# Autodesk Inventor assembly: złożenie ujoint
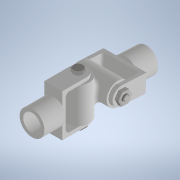
[picture p0: Inventor's stored thumbnail of the model, 180x180]
Saved by Autodesk Inventor 2021 (Build 250183000, 183)
## iProperties
Created: 2022-04-15
Part Number: złożenie ujoint
Document SubType Name: Assembly
Designer: Łukasz
Author: Łukasz
## Documents named in this file (7)
- E:\Pliki inventor i stl\motion platform\złożenie ujoint.iam
- E:\Pliki inventor i stl\motion platform\uJoint.1.ipt
- C:\Users\Łukasz\Documents\Inventor\Content Center Files\R2021\en-US\BS 292 (I)\BS 292 Part 1 - 6000 - 10 x 26 x 8.ipt
- E:\Pliki inventor i stl\motion platform\krzyżak.ipt
- C:\Users\Łukasz\Documents\Inventor\Content Center Files\R2021\en-US\AS 1110\AS 1110 - M8 x 65.ipt
- C:\Users\Łukasz\Documents\Inventor\Content Center Files\R2021\en-US\AS 1110\AS 1110 - M8 x 12.ipt
- C:\Users\Łukasz\Documents\Inventor\Content Center Files\R2021\en-US\AS 1474(1)\AS 1474 - M10(1).ipt
## Components (12 placed, 6 different names)
1. uJoint.1:1 — Rotational:2, Mate:1, Mate:2, Rigid:6
2. BS 292: Part 1 (I) (Metric) 6000 - 10 x 26 x 8:1 — Rigid:2, Rotational:2
3. BS 292: Part 1 (I) (Metric) 6000 - 10 x 26 x 8:2 — Rigid:3
4. BS 292: Part 1 (I) (Metric) 6000 - 10 x 26 x 8:3 — Rigid:1
5. BS 292: Part 1 (I) (Metric) 6000 - 10 x 26 x 8:4 — Rigid:4, Rotational:1
6. uJoint.1:2 — Rotational:1, Insert:1, Rigid:5
7. krzyżak:1 — Rigid:1, Rigid:2, Rigid:3, Rigid:4
8. AS 1110 - Metric M8 x 65:1 — Mate:1, Mate:2
9. AS 1474 - Metric M10:1 — Rigid:5
10. AS 1474 - Metric M10:2 — Rigid:6
11. AS 1110 - Metric M8 x 12:1 — Insert:1
12. AS 1110 - Metric M8 x 12:2
## Component patterns: (2 elements, first: AS 1110 - Metric M8 x 12:1)
## Relationships (11: WeldJoint 6, RevoluteJoint 2, Mate 2, Insert 1)
- Rigid:1 [WeldJoint]: BS 292: Part 1 (I) (Metric) 6000 - 10 x 26 x 8:3 ↔ krzyżak:1
- Rigid:2 [WeldJoint]: BS 292: Part 1 (I) (Metric) 6000 - 10 x 26 x 8:1 ↔ krzyżak:1
- Rigid:3 [WeldJoint]: BS 292: Part 1 (I) (Metric) 6000 - 10 x 26 x 8:2 ↔ krzyżak:1
- Rigid:4 [WeldJoint]: BS 292: Part 1 (I) (Metric) 6000 - 10 x 26 x 8:4 ↔ krzyżak:1
- Rotational:1 [RevoluteJoint]: BS 292: Part 1 (I) (Metric) 6000 - 10 x 26 x 8:4 ↔ uJoint.1:2
- Rotational:2 [RevoluteJoint]: uJoint.1:1 ↔ BS 292: Part 1 (I) (Metric) 6000 - 10 x 26 x 8:1
- Mate:1: uJoint.1:1 ↔ AS 1110 - Metric M8 x 65:1
- Mate:2: uJoint.1:1 ↔ AS 1110 - Metric M8 x 65:1
- Insert:1: uJoint.1:2 ↔ AS 1110 - Metric M8 x 12:1
- Rigid:5 [WeldJoint]: uJoint.1:2 ↔ AS 1474 - Metric M10:1
- Rigid:6 [WeldJoint]: uJoint.1:1 ↔ AS 1474 - Metric M10:2
